# Autodesk Inventor assembly: model_awds
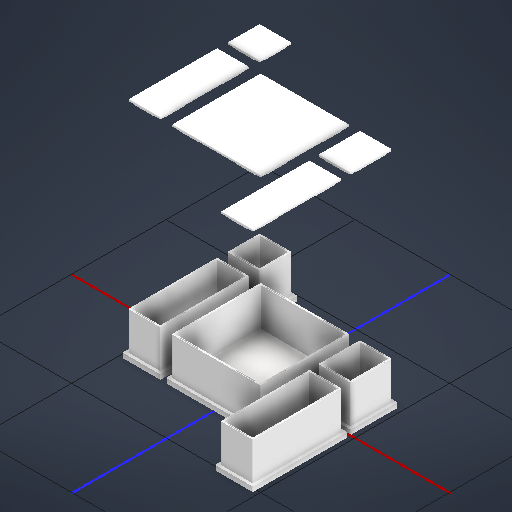
[picture p0: Inventor's stored thumbnail of the model, 512x512]
Saved by Autodesk Inventor 2025.2 (Build 292293000, 293)
## iProperties
Created: 2025-08-04
Part Number: model_awds
Document SubType Name: Assembly
Designer: sam
Author: sam
## Documents named in this file (9)
- G:\projects\primary\auto-water-distribution-system\model\assembly\model_awds.iam
- G:\projects\primary\auto-water-distribution-system\model\assembly\parts\block_main.ipt
- G:\projects\primary\auto-water-distribution-system\model\assembly\parts\block_main-lid.ipt
- G:\projects\primary\auto-water-distribution-system\model\assembly\parts\block_water-pipe.ipt
- G:\projects\primary\auto-water-distribution-system\model\assembly\parts\block_water-pipe_lid.ipt
- G:\projects\primary\auto-water-distribution-system\model\assembly\parts\block_pump.ipt
- G:\projects\primary\auto-water-distribution-system\model\assembly\parts\block_pump_lid.ipt
- G:\projects\primary\auto-water-distribution-system\model\assembly\parts\block_pump-connections.ipt
- G:\projects\primary\auto-water-distribution-system\model\assembly\parts\block_pump-connections_lid.ipt
## Components (10 placed, 8 different names)
1. block_main:1 — Flush:3, Mate:4, Mate:5, Flush:4, Flush:5, Flush:6
2. block_main-lid:1 — Mate:4, Mate:5, Flush:7, Flush:8, Flush:9, Flush:10
3. block_water-pipe:1 — Mate:2, Mate:3, Flush:3
4. block_water-pipe_lid:1 — Mate:2, Mate:3, Flush:8
5. block_pump:1 — Flush:4, Mate:6, Mate:7
6. block_pump_lid:1 — Mate:6, Mate:7, Flush:9
7. block_pump-connections:1 — Flush:5, Mate:8, Mate:9
8. block_pump-connections_lid:1 — Mate:8, Mate:9, Flush:10
9. block_water-pipe:2 — Flush:6
10. block_water-pipe_lid:2 — Flush:7
## Relationships (18: Mate 10, Flush 8)
- Mate:2: block_water-pipe:1 ↔ block_water-pipe_lid:1
- Mate:3: block_water-pipe:1 ↔ block_water-pipe_lid:1
- Flush:3: block_main:1 ↔ block_water-pipe:1
- Mate:4: block_main:1 ↔ block_main-lid:1
- Mate:5: block_main:1 ↔ block_main-lid:1
- Flush:4: block_main:1 ↔ block_pump:1
- Mate:6: block_pump:1 ↔ block_pump_lid:1
- Mate:7: block_pump:1 ↔ block_pump_lid:1
- Flush:5: block_main:1 ↔ block_pump-connections:1
- Mate:8: block_pump-connections:1 ↔ block_pump-connections_lid:1
- Mate:9: block_pump-connections:1 ↔ block_pump-connections_lid:1
- [Mate]: block_water-pipe:2 ↔ block_water-pipe_lid:2
- [Mate]: block_water-pipe:2 ↔ block_water-pipe_lid:2
- Flush:6: block_main:1 ↔ block_water-pipe:2
- Flush:7: block_main-lid:1 ↔ block_water-pipe_lid:2
- Flush:8: block_main-lid:1 ↔ block_water-pipe_lid:1
- Flush:9: block_main-lid:1 ↔ block_pump_lid:1
- Flush:10: block_main-lid:1 ↔ block_pump-connections_lid:1
## Named parameters: d17_d6 = 0 mm, d18_d7 = 0 mm
